# Autodesk Inventor assembly: ClawPart
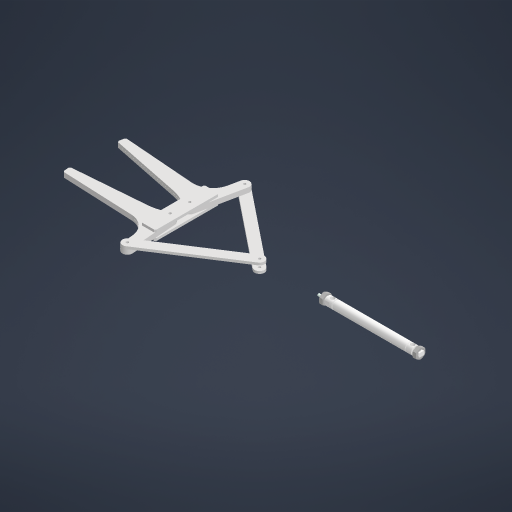
[picture p0: Inventor's stored thumbnail of the model, 512x512]
Saved by Autodesk Inventor 2023 (Build 270158000, 158)
## iProperties
Created: 2023-01-27
Part Number: ClawPart
Document SubType Name: Assembly
Designer: Terrence
Author: Terrence
## Documents named in this file (5)
- C:\Users\Terrence\Documents\FRC Long\ClawPart.iam
- C:\Users\Terrence\Documents\FRC Long\Solid1.ipt
- C:\Users\Terrence\Documents\FRC Long\Solid2.ipt
- C:\Users\Terrence\Documents\FRC Long\Solid3.ipt
- C:\Users\Terrence\Downloads\am-2034_6.iam
## Components (9 placed, 4 different names)
1. Solid1:1 — Insert:3, Mate:1, Mate:2, Insert:12
2. Solid2:1 — Insert:9, Insert:10
3. Solid3:1 — Insert:12, Insert:13
4. Solid2:2 — Insert:3, Insert:4
5. Solid1:2 — Insert:4, Mate:3, Mate:4
6. Solid3:2 — Insert:11, Insert:13
7. Solid1:3 — Mate:1, Mate:2, Insert:9
8. Solid1:5 — Mate:3, Mate:4, Insert:10, Insert:11
9. am-2034_6:1 [sub-assembly]
## Relationships (11: Insert 7, Mate 4)
- Insert:3: Solid1:1 ↔ Solid2:2
- Insert:4: Solid2:2 ↔ Solid1:2
- Mate:1: Solid1:1 ↔ Solid1:3
- Mate:2: Solid1:1 ↔ Solid1:3
- Mate:3: Solid1:2 ↔ Solid1:5
- Mate:4: Solid1:2 ↔ Solid1:5
- Insert:9: Solid2:1 ↔ Solid1:3
- Insert:10: Solid2:1 ↔ Solid1:5
- Insert:11: Solid3:2 ↔ Solid1:5
- Insert:12: Solid1:1 ↔ Solid3:1
- Insert:13 (12.7 mm): Solid3:1 ↔ Solid3:2
